# Autodesk Inventor assembly: Assembly3
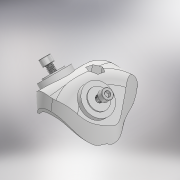
[picture p0: Inventor's stored thumbnail of the model, 180x180]
Saved by Autodesk Inventor 2021 (Build 250183000, 183)
## iProperties
Created: 2020-06-24
Part Number: Assembly3
Document SubType Name: Assembly
Designer: Derm
Author: Derm
## Documents named in this file (9)
- C:\Users\Derm\n95\v7\maskBodyV4Molds\Assembly3.iam
- C:\Users\Derm\n95\v7\maskBodyV4Molds\lowerWithoutPos.ipt
- C:\Users\Derm\n95\v7\maskBodyV4Molds\mainInnerPos.ipt
- C:\Users\Derm\n95\v7\maskBodyV4Molds\upper.ipt
- C:\Users\Derm\n95\v7\maskBodyV4Molds\pourTool.ipt
- C:\Users\Derm\n95\v7\maskBodyV4Molds\91290A211_BLACK-OXIDE CLASS 12.9 SOCKET HEAD CAP SCREW.ipt
- C:\Users\Derm\n95\v7\maskBodyV4Molds\90592A022_STEEL HEX NUT.ipt
- C:\Users\Derm\n95\v7\maskBodyV4Molds\main.ipt
- C:\Users\Derm\n95\v7\maskBodyV4Molds\innerPosPlug1.ipt
## Components (10 placed, 8 different names)
1. lowerWithoutPos:1 — Flush:1, Flush:2, Flush:3, Flush:4, Flush:5, Flush:6, Mate:5, Mate:7
2. mainInnerPos:1 — Flush:1, Flush:2, Flush:5, Flush:9, Flush:10
3. upper:1 — Flush:3, Flush:4, Flush:6, Flush:7, Mate:1, Mate:2, Mate:3
4. pourTool:1 — Flush:7, Mate:1
5. 91290A211_BLACK-OXIDE CLASS 12.9 SOCKET HEAD CAP SCREW:1 — Mate:2, Mate:6
6. 91290A211_BLACK-OXIDE CLASS 12.9 SOCKET HEAD CAP SCREW:2 — Mate:3, Mate:4
7. 90592A022_STEEL HEX NUT:1 — Mate:4, Mate:5
8. 90592A022_STEEL HEX NUT:2 — Mate:6, Mate:7
9. main:1 — Flush:9
10. innerPosPlug1:1 — Flush:10
## Relationships (16: Flush 9, Mate 7)
- Flush:1: lowerWithoutPos:1 ↔ mainInnerPos:1
- Flush:2: lowerWithoutPos:1 ↔ mainInnerPos:1
- Flush:3: lowerWithoutPos:1 ↔ upper:1
- Flush:4: lowerWithoutPos:1 ↔ upper:1
- Flush:5: lowerWithoutPos:1 ↔ mainInnerPos:1
- Flush:6: lowerWithoutPos:1 ↔ upper:1
- Flush:7: upper:1 ↔ pourTool:1
- Mate:1: upper:1 ↔ pourTool:1
- Mate:2: upper:1 ↔ 91290A211_BLACK-OXIDE CLASS 12.9 SOCKET HEAD CAP SCREW:1
- Mate:3: upper:1 ↔ 91290A211_BLACK-OXIDE CLASS 12.9 SOCKET HEAD CAP SCREW:2
- Mate:4: 91290A211_BLACK-OXIDE CLASS 12.9 SOCKET HEAD CAP SCREW:2 ↔ 90592A022_STEEL HEX NUT:1
- Mate:5: lowerWithoutPos:1 ↔ 90592A022_STEEL HEX NUT:1
- Mate:6: 91290A211_BLACK-OXIDE CLASS 12.9 SOCKET HEAD CAP SCREW:1 ↔ 90592A022_STEEL HEX NUT:2
- Mate:7: lowerWithoutPos:1 ↔ 90592A022_STEEL HEX NUT:2
- Flush:9: mainInnerPos:1 ↔ main:1
- Flush:10: mainInnerPos:1 ↔ innerPosPlug1:1
